# Autodesk Inventor assembly: Disceep32
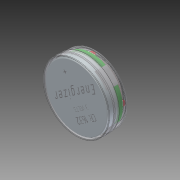
[picture p0: Inventor's stored thumbnail of the model, 180x180]
Saved by Autodesk Inventor 2014 (Build 180170000, 170)
## iProperties
Created: 2014-10-10
Part Number: Disceep32
Document SubType Name: Assembly
Designer: DV
Author: DV
## Documents named in this file (11)
- C:\Users\DV\Documents\github\Disceep\Disceep32.iam
- C:\Users\DV\Downloads\battery-cr1632.snapshot.2\Imported Components\bateriaCR1632-napisy\bateriaCR1632-napisy.ipt
- C:\Users\DV\Documents\github\Allegro_Design_Library\PCB.ipt
- C:\Users\DV\Documents\github\Allegro_Design_Library\NegBattTerminal.ipt
- C:\Users\DV\Documents\github\Allegro_Design_Library\PosBatClip.ipt
- C:\Users\DV\Documents\github\Disceep\12mmPiezo.ipt
- C:\Users\DV\Downloads\Imported Components\User Library-QUARTER\User Library-QUARTER.ipt
- C:\Users\DV\Downloads\User Library-LTST-C190EKT (1)\Imported Components\User Library-LTST-C190EKT\Assembly2.iam
- C:\Users\DV\Documents\github\Disceep\Case.ipt
- C:\Users\DV\Documents\github\Disceep\TSSOP_14.iam
- C:\Users\DV\Documents\github\Disceep\CaseBottom.ipt
## Components (16 placed, 10 different names)
1. bateriaCR1632-napisy:1 — Flush:1, Mate:3
2. PCB:1 — Flush:1, Mate:1, Mate:2, Tangent:1, Mate:4, Tangent:2, Mate:5, Mate:6, Tangent:3, Mate:7, Tangent:4, Mate:12, Mate:13, Mate:14, Mate:15
3. NegBattTerminal:1 — Flush:2, Mate:2
4. PosBatClip:1 — Tangent:1, Mate:4, Mate:8, Angle:1
5. PosBatClip:3 — Mate:6, Tangent:3, Mate:9
6. PosBatClip:2 — Tangent:2, Mate:5, Mate:8
7. PosBatClip:4 — Mate:7, Tangent:4, Mate:9, Angle:1
8. 12mmPiezo:1 — Flush:3, Mate:11, Mate:12
9. User Library-QUARTER:1
10. TSSOP_14:1 [sub-assembly] — Mate:15
11. Case:1 — Flush:4, Flush:5
12. CaseBottom:1 — Flush:5
13. Assembly2:1 [sub-assembly] — Mate:13, Mate:14
14. Assembly2:2 [sub-assembly]
15. Assembly2:3 [sub-assembly]
16. Assembly2:4 [sub-assembly]
## Component patterns: (4 elements, first: Assembly2:1)
## Relationships (24: Mate 14, Flush 5, Tangent 4, Angle 1)
- Flush:1 (-0.2 mm): bateriaCR1632-napisy:1 ↔ PCB:1
- Mate:1: PCB:1
- Flush:2: NegBattTerminal:1
- Mate:2: PCB:1 ↔ NegBattTerminal:1
- Mate:3: bateriaCR1632-napisy:1
- Tangent:1: PCB:1 ↔ PosBatClip:1
- Mate:4: PCB:1 ↔ PosBatClip:1
- Tangent:2: PCB:1 ↔ PosBatClip:2
- Mate:5: PCB:1 ↔ PosBatClip:2
- Mate:6: PCB:1 ↔ PosBatClip:3
- Tangent:3: PCB:1 ↔ PosBatClip:3
- Mate:7: PCB:1 ↔ PosBatClip:4
- Tangent:4: PCB:1 ↔ PosBatClip:4
- Mate:8: PosBatClip:1 ↔ PosBatClip:2
- Mate:9: PosBatClip:3 ↔ PosBatClip:4
- Angle:1 (90 deg): PosBatClip:1 ↔ PosBatClip:4
- Flush:3: 12mmPiezo:1
- Mate:11: 12mmPiezo:1
- Mate:12 (1.778 mm): PCB:1 ↔ 12mmPiezo:1
- Mate:13: PCB:1 ↔ Assembly2:1
- Mate:14 (6.858 mm): PCB:1 ↔ Assembly2:1
- Mate:15: PCB:1 ↔ TSSOP_14:1
- Flush:4: Case:1
- Flush:5: Case:1 ↔ CaseBottom:1
